# Autodesk Inventor assembly: DART 12 Lead Screw Module
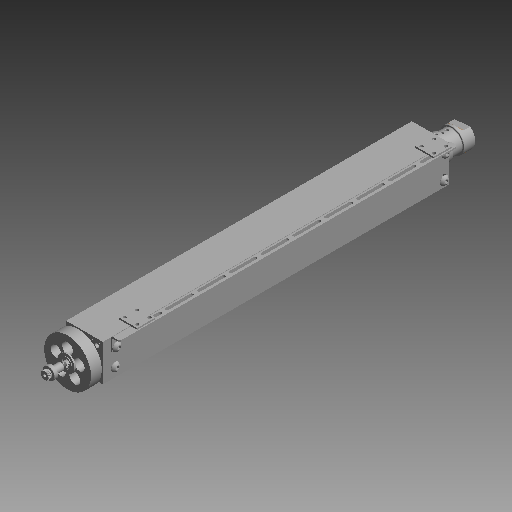
[picture p0: Inventor's stored thumbnail of the model, 512x512]
Saved by Autodesk Inventor 2017 (Build 210142000, 142)
## iProperties
Created: 2016-01-05
Part Number: DART 12 Lead Screw Module
Document SubType Name: Assembly
Designer: steele
Author: steele
Revision Number: ANY
## Documents named in this file (21)
- C:\snobotics\CAD-Development\robSteele\SnoBotics2016\DART 12inch from AM\DART 12 Lead Screw Module.iam
- C:\snobotics\CAD-Development\robSteele\SnoBotics2016\DART 12inch from AM\am-3260 Spacer.ipt
- C:\snobotics\CAD-Development\robSteele\SnoBotics2016\DART 12inch from AM\am-3254 DART 12 Square Tube Rev1-1.ipt
- C:\snobotics\CAD-Development\robSteele\SnoBotics2016\DART 12inch from AM\am-3253 DART Bearing Block.ipt
- C:\snobotics\CAD-Development\robSteele\SnoBotics2016\DART 12inch from AM\am-3259 DART Ram End Bearing.ipt
- C:\snobotics\CAD-Development\robSteele\SnoBotics2016\DART 12inch from AM\am-3257 DART 12 Lead Screw.ipt
- C:\snobotics\CAD-Development\robSteele\SnoBotics2016\DART 12inch from AM\am-3268 Gear, 14T, 48dp, Steel.ipt
- C:\snobotics\CAD-Development\robSteele\SnoBotics2016\DART 12inch from AM\am-3252 DART 12 Sensor Bracket.ipt
- C:\snobotics\CAD-Development\robSteele\SnoBotics2016\DART 12inch from AM\am-3258 DART Ram Cap.ipt
- C:\snobotics\CAD-Development\robSteele\SnoBotics2016\DART 12inch from AM\am-3256 DART Ram 12 Tube.ipt
- C:\snobotics\CAD-Development\robSteele\SnoBotics2016\DART 12inch from AM\am-3265 30T Pulley.ipt
- C:\snobotics\CAD-Development\robSteele\SnoBotics2016\DART 12inch from AM\am-1121.ipt
- C:\snobotics\CAD-Development\robSteele\SnoBotics2016\DART 12inch from AM\R3 Bearing.ipt
- C:\snobotics\CAD-Development\robSteele\SnoBotics2016\DART 12inch from AM\Retaining Ring 3125_97431A310.ipt
- C:\snobotics\CAD-Development\robSteele\SnoBotics2016\DART 12inch from AM\am-3255 DART Back Bearing.ipt
- C:\snobotics\CAD-Development\robSteele\SnoBotics2016\DART 12inch from AM\am-3262 DART Nut.ipt
- C:\snobotics\CAD-Development\robSteele\SnoBotics2016\DART 12inch from AM\1614Z Bearing_smart.ipt
- C:\snobotics\CAD-Development\robSteele\SnoBotics2016\DART 12inch from AM\5-16 washer.ipt
- C:\snobotics\CAD-Development\robSteele\SnoBotics2016\DART 12inch from AM\1875 dia 500 long 8-32_91259A166.ipt
- C:\snobotics\CAD-Development\robSteele\SnoBotics2016\DART 12inch from AM\Hall Effect Sensor.ipt
- C:\snobotics\CAD-Development\robSteele\SnoBotics2016\DART 12inch from AM\BHCS 10-32 x 0.375 phillips_SBHCSCREW 0.19-32x0.5-HX-C.ipt
## Components (33 placed, 33 different names)
1. am-3260 Spacer_3
2. am-3260 Spacer_4
3. am-3254 DART 12 Square Tube Rev1-1_5
4. am-3253 DART Bearing Block_6
5. am-3259 DART Ram End Bearing_7
6. am-3257 DART 12 Lead Screw_8 — Insert:2, Mate:2
7. am-3268 Gear, 14T, 48dp, Steel_9
8. am-3252 DART 12 Sensor Bracket_10
9. am-3258 DART Ram Cap_11 — Mate:2
10. am-3256 DART Ram 12 Tube_12
11. am-3265 30T Pulley_13
12. am-1121_14
13. R3 Bearing_15
14. Retaining Ring 3125_97431A310_16
15. Retaining Ring 3125_97431A310_17
16. am-3255 DART Back Bearing_18
17. am-3262 DART Nut_19 — Insert:2
18. 1614Z Bearing_smart_20
19. 1614Z Bearing_smart_21
20. 5-16 washer_22
21. 5-16 washer_23
22. 1875 dia 500 long 8-32_91259A166_24
23. Hall Effect Sensor_25
24. am-3255 DART Back Bearing_26
25. Hall Effect Sensor_27
26. BHCS 10-32 x 0.375 phillips_SBHCSCREW 0.19-32x0.5-HX-C_28
27. BHCS 10-32 x 0.375 phillips_SBHCSCREW 0.19-32x0.5-HX-C_29
28. BHCS 10-32 x 0.375 phillips_SBHCSCREW 0.19-32x0.5-HX-C_30
29. BHCS 10-32 x 0.375 phillips_SBHCSCREW 0.19-32x0.5-HX-C_31
30. BHCS 10-32 x 0.375 phillips_SBHCSCREW 0.19-32x0.5-HX-C_32
31. BHCS 10-32 x 0.375 phillips_SBHCSCREW 0.19-32x0.5-HX-C_33
32. BHCS 10-32 x 0.375 phillips_SBHCSCREW 0.19-32x0.5-HX-C_34
33. BHCS 10-32 x 0.375 phillips_SBHCSCREW 0.19-32x0.5-HX-C_35
## Relationships (2: Insert 1, Mate 1)
- Insert:2: am-3257 DART 12 Lead Screw_8 ↔ am-3262 DART Nut_19
- Mate:2: am-3257 DART 12 Lead Screw_8 ↔ am-3258 DART Ram Cap_11
